# Autodesk Inventor assembly: KTN_MultiPass_actual_distances_sizes_configs
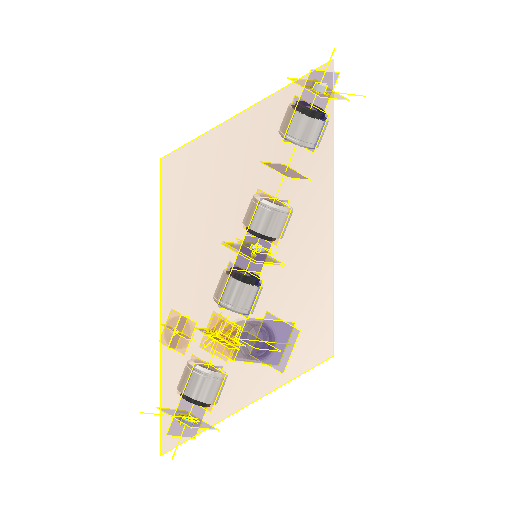
[picture p0: Inventor's stored thumbnail of the model, 512x512]
Saved by Autodesk Inventor 2026.1 (Build 301233000, 233)
## iProperties
Created: 2024-04-24
Part Number: KTN_MultiPass_actual_distances_sizes_configs
Document SubType Name: Assembly
Designer: kerlin
Author: kerlin
## Documents named in this file (8)
- C:\Users\farin012\Downloads\fig4\fig4\KTN_MultiPass_actual_distances_sizes_configs.iam
- C:\Users\farin012\Downloads\fig4\fig4\LSM03-BB-Solidworks.ipt
- C:\Users\farin012\Downloads\fig4\fig4\ExitMirror.ipt
- C:\Users\farin012\Downloads\fig4\fig4\Lens.ipt
- C:\Users\farin012\Downloads\fig4\fig4\EntryMirror.ipt
- C:\Users\farin012\Downloads\fig4\fig4\pckngo_D1\3x4x1p2_KTN.ipt
- C:\Users\farin012\Downloads\fig4\fig4\latest_cylindrical_10x12_LK1982L1.ipt
- C:\Users\farin012\Downloads\fig4\fig4\BB05-E03-Solidworks\BB05-E03-Solidworks\BB05-E03-Solidworks.ipt
## Components (12 placed, 7 different names)
1. LSM03-BB-Solidworks:1 — Mate:3, Mate:4, Mate:17, Mate:21, Mate:24, Mate:25, Mate:26, Mate:39
2. LSM03-BB-Solidworks:2 — Mate:3, Mate:17, Mate:31, Mate:32, Mate:42
3. LSM03-BB-Solidworks:3 — Mate:1, Mate:18, Mate:27, Mate:33, Mate:38, Mate:40
4. LSM03-BB-Solidworks:4 — Mate:1, Mate:4, Mate:18, Mate:23, Mate:34, Mate:35, Mate:36, Mate:41
5. ExitMirror:1 — Mate:34, Mate:35, Flush:13, Flush:15
6. Lens:1 — Flush:20, Mate:43, Mate:44
7. EntryMirror:1 — Flush:13, Flush:14, Mate:36, Flush:20, Mate:44
8. 3x4x1p2_KTN:1 — Mate:21, Mate:22, Mate:23, Flush:12
9. latest_cylindrical_10x12_LK1982L1:1 — Mate:24, Mate:25, Flush:12, Mate:26
10. LSM03-BB-Solidworks:5 — Flush:15, Mate:37, Mate:38
11. BB05-E03-Solidworks:1 — Mate:27, Mate:28, Mate:33
12. BB05-E03-Solidworks:2 — Mate:30, Mate:31, Mate:32
## Relationships (33: Mate 28, Flush 5)
- Mate:1: LSM03-BB-Solidworks:3 ↔ LSM03-BB-Solidworks:4
- Mate:3: LSM03-BB-Solidworks:1 ↔ LSM03-BB-Solidworks:2
- Mate:4: LSM03-BB-Solidworks:1 ↔ LSM03-BB-Solidworks:4
- Mate:17: LSM03-BB-Solidworks:1 ↔ LSM03-BB-Solidworks:2
- Mate:18: LSM03-BB-Solidworks:3 ↔ LSM03-BB-Solidworks:4
- Mate:21: LSM03-BB-Solidworks:1 ↔ 3x4x1p2_KTN:1
- Mate:22: 3x4x1p2_KTN:1
- Mate:23 (19.1 mm): LSM03-BB-Solidworks:4 ↔ 3x4x1p2_KTN:1
- Mate:24: LSM03-BB-Solidworks:1 ↔ latest_cylindrical_10x12_LK1982L1:1
- Mate:25: LSM03-BB-Solidworks:1 ↔ latest_cylindrical_10x12_LK1982L1:1
- Flush:12 (-2.885 mm): 3x4x1p2_KTN:1 ↔ latest_cylindrical_10x12_LK1982L1:1
- Mate:26 (15.5 mm): LSM03-BB-Solidworks:1 ↔ latest_cylindrical_10x12_LK1982L1:1
- Mate:27: LSM03-BB-Solidworks:3 ↔ BB05-E03-Solidworks:1
- Mate:28: BB05-E03-Solidworks:1
- Mate:30: BB05-E03-Solidworks:2
- Mate:31: LSM03-BB-Solidworks:2 ↔ BB05-E03-Solidworks:2
- Mate:32 (18.89 mm): LSM03-BB-Solidworks:2 ↔ BB05-E03-Solidworks:2
- Mate:33 (18.89 mm): LSM03-BB-Solidworks:3 ↔ BB05-E03-Solidworks:1
- Mate:34: LSM03-BB-Solidworks:4 ↔ ExitMirror:1
- Mate:35: LSM03-BB-Solidworks:4 ↔ ExitMirror:1
- Flush:13 (-4.5 mm): ExitMirror:1 ↔ EntryMirror:1
- Flush:14: EntryMirror:1
- Mate:36: LSM03-BB-Solidworks:4 ↔ EntryMirror:1
- Flush:15: ExitMirror:1 ↔ LSM03-BB-Solidworks:5
- Flush:20 (-50 mm): Lens:1 ↔ EntryMirror:1
- Mate:37: LSM03-BB-Solidworks:5
- Mate:38: LSM03-BB-Solidworks:3 ↔ LSM03-BB-Solidworks:5
- Mate:39: LSM03-BB-Solidworks:1
- Mate:40: LSM03-BB-Solidworks:3
- Mate:41: LSM03-BB-Solidworks:4
- Mate:42: LSM03-BB-Solidworks:2
- Mate:43: Lens:1
- Mate:44: Lens:1 ↔ EntryMirror:1
